# Autodesk Inventor assembly: centre wing
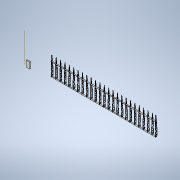
[picture p0: Inventor's stored thumbnail of the model, 180x180]
Saved by Autodesk Inventor 2022 (Build 260153000, 153)
## iProperties
Created: 2021-03-09
Part Number: centre wing
Document SubType Name: Assembly
Designer: Ferdinand Hubbard
Author: Ferdinand Hubbard
## Documents named in this file (6)
- C:\Users\Ferdinand Hubbard\Desktop\solar-plane\cad\centre wing section.iam
- C:\Users\Ferdinand Hubbard\Desktop\solar-plane\cad\18mm tube.ipt
- C:\Users\Ferdinand Hubbard\Desktop\solar-plane\cad\15mm tube.ipt
- C:\Users\Ferdinand Hubbard\Desktop\solar-plane\cad\airfoils\full airfoil\full airfoil blueprint 19 mm.ipt
- C:\Users\Ferdinand Hubbard\Desktop\solar-plane\cad\airfoils\full airfoil\full airfoil blueprint 16 mm.ipt
- C:\Users\Ferdinand Hubbard\Desktop\solar-plane\cad\6 cell pack.ipt
## Components (34 placed, 5 different names)
1. 18mm tube:2 — Mate:1, Mate:2, Mate:5, Mate:6
2. 15mm tube:2 — Mate:1, Mate:2, Mate:14, Flush:1, Mate:17, Mate:84
3. 18mm tube:3 — Mate:15, Flush:3
4. 15mm tube:3 — Mate:5, Mate:6
5. 18mm tube:4
6. 15mm tube:4 — Mate:13, Flush:2, Mate:83
7. 18mm tube:5 — Flush:4, Mate:16
8. 15mm tube:5
9. full airfoil blueprint 19 mm:2 — Mate:15, Flush:3, Flush:4, Mate:16
10. full airfoil blueprint 16 mm:2 — Mate:13, Mate:14, Flush:1, Flush:2, Mate:18
11. 6 cell pack:1
12. full airfoil blueprint 16 mm:3 — Mate:17, Mate:18, Mate:64
13. full airfoil blueprint 16 mm:4 — Mate:19, Mate:20, Mate:21, Mate:25, Mate:26, Mate:27
14. full airfoil blueprint 16 mm:5 — Mate:19, Mate:20, Mate:21, Mate:64, Mate:83, Mate:84
15. full airfoil blueprint 16 mm:6 — Mate:37, Mate:38, Mate:39
16. full airfoil blueprint 16 mm:7 — Mate:25, Mate:26, Mate:27
17. full airfoil blueprint 16 mm:8
18. full airfoil blueprint 16 mm:9 — Mate:37, Mate:38, Mate:39
19. full airfoil blueprint 16 mm:10 — Mate:61, Mate:62, Mate:63
20. full airfoil blueprint 16 mm:11
21. full airfoil blueprint 16 mm:12
22. full airfoil blueprint 16 mm:13 — Mate:61, Mate:62, Mate:63
23. full airfoil blueprint 16 mm:14
24. full airfoil blueprint 16 mm:15
25. full airfoil blueprint 16 mm:16
26. full airfoil blueprint 16 mm:17
27. full airfoil blueprint 16 mm:18 — Mate:80, Mate:81, Mate:82
28. full airfoil blueprint 16 mm:19
29. full airfoil blueprint 16 mm:20
30. full airfoil blueprint 16 mm:21 — Mate:80, Mate:81, Mate:82
31. full airfoil blueprint 16 mm:22
32. full airfoil blueprint 16 mm:23
33. full airfoil blueprint 16 mm:24
34. full airfoil blueprint 16 mm:25
## Relationships (88: Mate 84, Flush 4)
- Mate:1: 18mm tube:2 ↔ 15mm tube:2
- Mate:2: 18mm tube:2 ↔ 15mm tube:2
- [Mate]: 18mm tube:3 ↔ 15mm tube:3
- [Mate]: 18mm tube:3 ↔ 15mm tube:3
- Mate:5: 18mm tube:2 ↔ 15mm tube:3
- Mate:6: 18mm tube:2 ↔ 15mm tube:3
- [Mate]: 18mm tube:4 ↔ 15mm tube:4
- [Mate]: 18mm tube:4 ↔ 15mm tube:4
- [Mate]: 18mm tube:5 ↔ 15mm tube:5
- [Mate]: 18mm tube:5 ↔ 15mm tube:5
- [Mate]: 18mm tube:4 ↔ 15mm tube:5
- [Mate]: 18mm tube:4 ↔ 15mm tube:5
- Mate:13: 15mm tube:4 ↔ full airfoil blueprint 16 mm:2
- Mate:14: 15mm tube:2 ↔ full airfoil blueprint 16 mm:2
- Flush:1 (12 mm): 15mm tube:2 ↔ full airfoil blueprint 16 mm:2
- Flush:2 (12 mm): 15mm tube:4 ↔ full airfoil blueprint 16 mm:2
- Mate:15: 18mm tube:3 ↔ full airfoil blueprint 19 mm:2
- Flush:3: 18mm tube:3 ↔ full airfoil blueprint 19 mm:2
- Flush:4: 18mm tube:5 ↔ full airfoil blueprint 19 mm:2
- Mate:16: 18mm tube:5 ↔ full airfoil blueprint 19 mm:2
- Mate:17: 15mm tube:2 ↔ full airfoil blueprint 16 mm:3
- Mate:18 (80 mm): full airfoil blueprint 16 mm:2 ↔ full airfoil blueprint 16 mm:3
- Mate:19: full airfoil blueprint 16 mm:4 ↔ full airfoil blueprint 16 mm:5
- Mate:20 (80 mm): full airfoil blueprint 16 mm:4 ↔ full airfoil blueprint 16 mm:5
- Mate:21: full airfoil blueprint 16 mm:4 ↔ full airfoil blueprint 16 mm:5
- [Mate]: full airfoil blueprint 16 mm:6 ↔ full airfoil blueprint 16 mm:7
- [Mate] (80 mm): full airfoil blueprint 16 mm:6 ↔ full airfoil blueprint 16 mm:7
- [Mate]: full airfoil blueprint 16 mm:6 ↔ full airfoil blueprint 16 mm:7
- Mate:25 (80 mm): full airfoil blueprint 16 mm:4 ↔ full airfoil blueprint 16 mm:7
- Mate:26: full airfoil blueprint 16 mm:4 ↔ full airfoil blueprint 16 mm:7
- Mate:27: full airfoil blueprint 16 mm:4 ↔ full airfoil blueprint 16 mm:7
- [Mate]: full airfoil blueprint 16 mm:8 ↔ full airfoil blueprint 16 mm:9
- [Mate] (80 mm): full airfoil blueprint 16 mm:8 ↔ full airfoil blueprint 16 mm:9
- [Mate]: full airfoil blueprint 16 mm:8 ↔ full airfoil blueprint 16 mm:9
- [Mate]: full airfoil blueprint 16 mm:10 ↔ full airfoil blueprint 16 mm:11
- [Mate] (80 mm): full airfoil blueprint 16 mm:10 ↔ full airfoil blueprint 16 mm:11
- [Mate]: full airfoil blueprint 16 mm:10 ↔ full airfoil blueprint 16 mm:11
- [Mate] (80 mm): full airfoil blueprint 16 mm:8 ↔ full airfoil blueprint 16 mm:11
- [Mate]: full airfoil blueprint 16 mm:8 ↔ full airfoil blueprint 16 mm:11
- [Mate]: full airfoil blueprint 16 mm:8 ↔ full airfoil blueprint 16 mm:11
- Mate:37 (80 mm): full airfoil blueprint 16 mm:6 ↔ full airfoil blueprint 16 mm:9
- Mate:38: full airfoil blueprint 16 mm:6 ↔ full airfoil blueprint 16 mm:9
- Mate:39: full airfoil blueprint 16 mm:6 ↔ full airfoil blueprint 16 mm:9
- [Mate]: full airfoil blueprint 16 mm:12 ↔ full airfoil blueprint 16 mm:13
- [Mate] (80 mm): full airfoil blueprint 16 mm:12 ↔ full airfoil blueprint 16 mm:13
- [Mate]: full airfoil blueprint 16 mm:12 ↔ full airfoil blueprint 16 mm:13
- [Mate]: full airfoil blueprint 16 mm:14 ↔ full airfoil blueprint 16 mm:15
- [Mate] (80 mm): full airfoil blueprint 16 mm:14 ↔ full airfoil blueprint 16 mm:15
- [Mate]: full airfoil blueprint 16 mm:14 ↔ full airfoil blueprint 16 mm:15
- [Mate] (80 mm): full airfoil blueprint 16 mm:12 ↔ full airfoil blueprint 16 mm:15
- [Mate]: full airfoil blueprint 16 mm:12 ↔ full airfoil blueprint 16 mm:15
- [Mate]: full airfoil blueprint 16 mm:12 ↔ full airfoil blueprint 16 mm:15
- [Mate]: full airfoil blueprint 16 mm:16 ↔ full airfoil blueprint 16 mm:17
- [Mate] (80 mm): full airfoil blueprint 16 mm:16 ↔ full airfoil blueprint 16 mm:17
- [Mate]: full airfoil blueprint 16 mm:16 ↔ full airfoil blueprint 16 mm:17
- [Mate]: full airfoil blueprint 16 mm:18 ↔ full airfoil blueprint 16 mm:19
- [Mate] (80 mm): full airfoil blueprint 16 mm:18 ↔ full airfoil blueprint 16 mm:19
- [Mate]: full airfoil blueprint 16 mm:18 ↔ full airfoil blueprint 16 mm:19
- [Mate] (80 mm): full airfoil blueprint 16 mm:16 ↔ full airfoil blueprint 16 mm:19
- [Mate]: full airfoil blueprint 16 mm:16 ↔ full airfoil blueprint 16 mm:19
- [Mate]: full airfoil blueprint 16 mm:16 ↔ full airfoil blueprint 16 mm:19
- [Mate] (80 mm): full airfoil blueprint 16 mm:14 ↔ full airfoil blueprint 16 mm:17
- [Mate]: full airfoil blueprint 16 mm:14 ↔ full airfoil blueprint 16 mm:17
- [Mate]: full airfoil blueprint 16 mm:14 ↔ full airfoil blueprint 16 mm:17
- Mate:61 (80 mm): full airfoil blueprint 16 mm:10 ↔ full airfoil blueprint 16 mm:13
- Mate:62: full airfoil blueprint 16 mm:10 ↔ full airfoil blueprint 16 mm:13
- Mate:63: full airfoil blueprint 16 mm:10 ↔ full airfoil blueprint 16 mm:13
- Mate:64 (80 mm): full airfoil blueprint 16 mm:3 ↔ full airfoil blueprint 16 mm:5
- [Mate]: full airfoil blueprint 16 mm:20 ↔ full airfoil blueprint 16 mm:21
- [Mate] (80 mm): full airfoil blueprint 16 mm:20 ↔ full airfoil blueprint 16 mm:21
- [Mate]: full airfoil blueprint 16 mm:20 ↔ full airfoil blueprint 16 mm:21
- [Mate]: full airfoil blueprint 16 mm:22 ↔ full airfoil blueprint 16 mm:23
- [Mate] (80 mm): full airfoil blueprint 16 mm:22 ↔ full airfoil blueprint 16 mm:23
- [Mate]: full airfoil blueprint 16 mm:22 ↔ full airfoil blueprint 16 mm:23
- [Mate]: full airfoil blueprint 16 mm:24 ↔ full airfoil blueprint 16 mm:25
- [Mate] (80 mm): full airfoil blueprint 16 mm:24 ↔ full airfoil blueprint 16 mm:25
- [Mate]: full airfoil blueprint 16 mm:24 ↔ full airfoil blueprint 16 mm:25
- [Mate] (80 mm): full airfoil blueprint 16 mm:22 ↔ full airfoil blueprint 16 mm:25
- [Mate]: full airfoil blueprint 16 mm:22 ↔ full airfoil blueprint 16 mm:25
- [Mate]: full airfoil blueprint 16 mm:22 ↔ full airfoil blueprint 16 mm:25
- [Mate] (80 mm): full airfoil blueprint 16 mm:20 ↔ full airfoil blueprint 16 mm:23
- [Mate]: full airfoil blueprint 16 mm:20 ↔ full airfoil blueprint 16 mm:23
- [Mate]: full airfoil blueprint 16 mm:20 ↔ full airfoil blueprint 16 mm:23
- Mate:80 (80 mm): full airfoil blueprint 16 mm:18 ↔ full airfoil blueprint 16 mm:21
- Mate:81: full airfoil blueprint 16 mm:18 ↔ full airfoil blueprint 16 mm:21
- Mate:82: full airfoil blueprint 16 mm:18 ↔ full airfoil blueprint 16 mm:21
- Mate:83: 15mm tube:4 ↔ full airfoil blueprint 16 mm:5
- Mate:84: 15mm tube:2 ↔ full airfoil blueprint 16 mm:5
## Named parameters: d99_d97 = 0 mm, d100_d98 = 0 mm, d103_d97 = 0 mm, d104_d98 = 0 mm, d105_d99_d97 = 0 mm, d106_d100_d98 = 0 mm, d107_d101 = 0 mm, d108_d102 = 0 mm, d146_d143 = 0 mm, d147_d144 = 80 mm, d148_d145 = 0 mm, d152_d143 = 0 mm, d153_d144 = 80 mm, d154_d145 = 0 mm, d155_d146_d143 = 0 mm, d156_d147_d144 = 80 mm, d157_d148_d145 = 0 mm, d158_d149 = 80 mm, d159_d150 = 0 mm, d160_d151 = 0 mm, d164_d143 = 0 mm, d165_d144 = 80 mm, d166_d145 = 0 mm, d167_d146_d143 = 0 mm, d168_d147_d144 = 80 mm, d169_d148_d145 = 0 mm, d170_d149 = 80 mm, d171_d150 = 0 mm, d172_d151 = 0 mm, d173_d152_d143 = 0 mm, d174_d153_d144 = 80 mm, d175_d154_d145 = 0 mm, d176_d155_d146_d143 = 0 mm, d177_d156_d147_d144 = 80 mm, d178_d157_d148_d145 = 0 mm, d179_d158_d149 = 80 mm, d180_d159_d150 = 0 mm, d181_d160_d151 = 0 mm, d182_d161 = 80 mm, d183_d162 = 0 mm, d184_d163 = 0 mm, d189_d167_d146_d143 = 0 mm, d190_d168_d147_d144 = 80 mm, d191_d169_d148_d145 = 0 mm, d192_d173_d152_d143 = 0 mm, d193_d174_d153_d144 = 80 mm, d194_d175_d154_d145 = 0 mm, d195_d176_d155_d146_d143 = 0 mm, d196_d177_d156_d147_d144 = 80 mm, d197_d178_d157_d148_d145 = 0 mm, d198_d179_d158_d149 = 80 mm, d199_d180_d159_d150 = 0 mm, d200_d181_d160_d151 = 0 mm, d201_d182_d161 = 80 mm, d202_d183_d162 = 0 mm, d203_d184_d163 = 0 mm
